# Autodesk Inventor assembly: ABEJA_COMPLETA
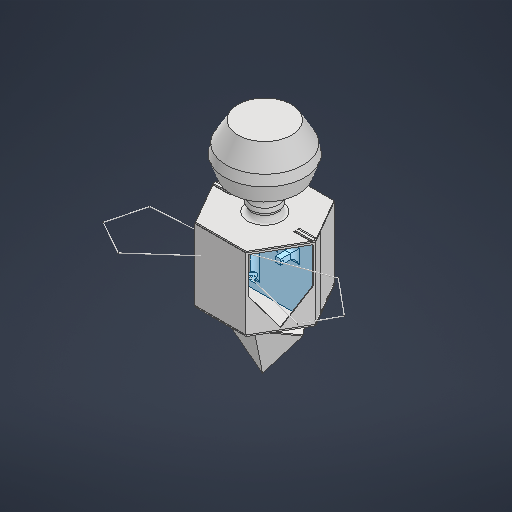
[picture p0: Inventor's stored thumbnail of the model, 512x512]
Saved by Autodesk Inventor 2026.2 (Build 302298000, 298)
## iProperties
Created: 2026-05-21
Part Number: ABEJA_COMPLETA
Document SubType Name: Assembly
Designer: juand
Author: juand
## Documents named in this file (13)
- C:\Users\juand\OneDrive - Universidad de los Andes\UNIANDES\6_SEMESTRE\DINAMICA_DE_MAQUINARIA\TALLER_3\la_abeja_mecanica\CAD_grande\ABEJA_COMPLETA.iam
- C:\Users\juand\OneDrive - Universidad de los Andes\UNIANDES\6_SEMESTRE\DINAMICA_DE_MAQUINARIA\TALLER_3\la_abeja_mecanica\CAD_grande\BASE_MECANISMO.ipt
- C:\Users\juand\OneDrive - Universidad de los Andes\UNIANDES\6_SEMESTRE\DINAMICA_DE_MAQUINARIA\TALLER_3\la_abeja_mecanica\CAD_grande\SERVO.ipt
- C:\Users\juand\OneDrive - Universidad de los Andes\UNIANDES\6_SEMESTRE\DINAMICA_DE_MAQUINARIA\TALLER_3\la_abeja_mecanica\CAD_grande\ESLABON_1.ipt
- C:\Users\juand\OneDrive - Universidad de los Andes\UNIANDES\6_SEMESTRE\DINAMICA_DE_MAQUINARIA\TALLER_3\la_abeja_mecanica\CAD_grande\ESLABON_2.ipt
- C:\Users\juand\OneDrive - Universidad de los Andes\UNIANDES\6_SEMESTRE\DINAMICA_DE_MAQUINARIA\TALLER_3\la_abeja_mecanica\CAD_grande\ESLABON_3.ipt
- C:\Users\juand\OneDrive - Universidad de los Andes\UNIANDES\6_SEMESTRE\DINAMICA_DE_MAQUINARIA\TALLER_3\la_abeja_mecanica\CAD_grande\carcasa_cuerpo_abeja.ipt
- C:\Users\juand\OneDrive - Universidad de los Andes\UNIANDES\6_SEMESTRE\DINAMICA_DE_MAQUINARIA\TALLER_3\la_abeja_mecanica\CAD_grande\tapa_cuerpo_abeja.ipt
- C:\Users\juand\OneDrive - Universidad de los Andes\UNIANDES\6_SEMESTRE\DINAMICA_DE_MAQUINARIA\TALLER_3\la_abeja_mecanica\CAD_grande\cola.ipt
- C:\Users\juand\OneDrive - Universidad de los Andes\UNIANDES\6_SEMESTRE\DINAMICA_DE_MAQUINARIA\TALLER_3\la_abeja_mecanica\CAD_grande\ala.ipt
- C:\Users\juand\OneDrive - Universidad de los Andes\UNIANDES\6_SEMESTRE\DINAMICA_DE_MAQUINARIA\TALLER_3\la_abeja_mecanica\CAD_grande\ala_MIR.ipt
- C:\Users\juand\OneDrive - Universidad de los Andes\UNIANDES\6_SEMESTRE\DINAMICA_DE_MAQUINARIA\TALLER_3\la_abeja_mecanica\CAD_grande\cabeza_1.ipt
- C:\Users\juand\OneDrive - Universidad de los Andes\UNIANDES\6_SEMESTRE\DINAMICA_DE_MAQUINARIA\TALLER_3\la_abeja_mecanica\CAD_grande\cabeza_2.ipt
## Components (13 placed, 12 different names)
1. BASE_MECANISMO:1 — Mate:1, Mate:2, Mate:3, Rotational:3, Mate:4, Flush:1, Cylindrical:2
2. SERVO:1 — Mate:1, Mate:2, Mate:3, Rotational:1
3. ESLABON_1:1 — Rotational:1, Rotational:2
4. ESLABON_2:1 — Rotational:2, Cylindrical:1, Ball:5, Ball:7
5. ESLABON_3:1 — Rotational:3, Cylindrical:1, Ball:6
6. carcasa_cuerpo_abeja:1 — Mate:4, Flush:1, Cylindrical:2, Mate:5, Flush:2, Flush:3, Mate:6, Flush:4, Flush:5
7. tapa_cuerpo_abeja:1 — Mate:5, Flush:2, Flush:3, Ball:8
8. tapa_cuerpo_abeja:2 — Mate:6, Flush:4, Flush:5, Ball:1
9. cola:1 — Ball:1
10. ala:1 — Ball:5, Ball:6
11. ala_MIR:1 — Ball:7
12. cabeza_1:1 — Rotational:4, Rotational:5
13. cabeza_2:1 — Rotational:4, Rotational:5, Ball:8
## Relationships (23: Mate 6, RevoluteJoint 5, Flush 5, BallJoint 5, CylindricalJoint 2)
- Mate:1: BASE_MECANISMO:1 ↔ SERVO:1
- Mate:2: BASE_MECANISMO:1 ↔ SERVO:1
- Mate:3: BASE_MECANISMO:1 ↔ SERVO:1
- Rotational:1 [RevoluteJoint]: SERVO:1 ↔ ESLABON_1:1
- Rotational:2 [RevoluteJoint]: ESLABON_1:1 ↔ ESLABON_2:1
- Rotational:3 [RevoluteJoint]: BASE_MECANISMO:1 ↔ ESLABON_3:1
- Cylindrical:1: ESLABON_2:1 ↔ ESLABON_3:1
- Mate:4: BASE_MECANISMO:1 ↔ carcasa_cuerpo_abeja:1
- Flush:1 (1.5 mm): BASE_MECANISMO:1 ↔ carcasa_cuerpo_abeja:1
- Cylindrical:2: BASE_MECANISMO:1 ↔ carcasa_cuerpo_abeja:1
- Mate:5: carcasa_cuerpo_abeja:1 ↔ tapa_cuerpo_abeja:1
- Flush:2: carcasa_cuerpo_abeja:1 ↔ tapa_cuerpo_abeja:1
- Flush:3: carcasa_cuerpo_abeja:1 ↔ tapa_cuerpo_abeja:1
- Mate:6: carcasa_cuerpo_abeja:1 ↔ tapa_cuerpo_abeja:2
- Flush:4: carcasa_cuerpo_abeja:1 ↔ tapa_cuerpo_abeja:2
- Flush:5: carcasa_cuerpo_abeja:1 ↔ tapa_cuerpo_abeja:2
- Ball:1: tapa_cuerpo_abeja:2 ↔ cola:1
- Ball:5: ESLABON_2:1 ↔ ala:1
- Ball:6: ESLABON_3:1 ↔ ala:1
- Ball:7: ESLABON_2:1 ↔ ala_MIR:1
- Rotational:4 [RevoluteJoint]: cabeza_1:1 ↔ cabeza_2:1
- Rotational:5 [RevoluteJoint]: cabeza_1:1 ↔ cabeza_2:1
- Ball:8: tapa_cuerpo_abeja:1 ↔ cabeza_2:1
